# Autodesk Inventor assembly: Threaded Rod Actuator
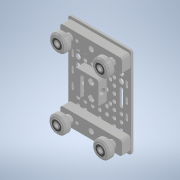
[picture p0: Inventor's stored thumbnail of the model, 180x180]
Saved by Autodesk Inventor 2020 (Build 240168000, 168)
## iProperties
Created: 2019-10-22
Part Number: Threaded Rod Actuator
Document SubType Name: Assembly
Designer: Johnson Ebenezer R
Author: Johnson Ebenezer R
## Documents named in this file (9)
- E:\My Tinkering Files\[2019-10-15][1330] Cam Controlled - PCB Paper's Fixture Hole - Punching Maching\Cam Controlled Paper Punching Machine (Prototype V2)\V-Slot Gantry Kit Universal (with gap for lead screw)\Gantry Kit (Vertical).iam
- E:\My Tinkering Files\[2019-10-15][1330] Cam Controlled - PCB Paper's Fixture Hole - Punching Maching\Cam Controlled Paper Punching Machine (Prototype V2)\V-Slot Gantry Kit Universal (with gap for lead screw)\V-Slot Gantry Plate 20-80mm.ipt
- E:\My Tinkering Files\[2019-10-15][1330] Cam Controlled - PCB Paper's Fixture Hole - Punching Maching\Cam Controlled Paper Punching Machine (Prototype V2)\V-Slot Gantry Kit Universal (with gap for lead screw)\8mm Acme Anti Backlash Nut Block.ipt
- E:\My Tinkering Files\[2019-10-15][1330] Cam Controlled - PCB Paper's Fixture Hole - Punching Maching\Cam Controlled Paper Punching Machine (Prototype V2)\V-Slot Gantry Kit Universal (with gap for lead screw)\Spacer Block.ipt
- E:\My Tinkering Files\[2019-10-15][1330] Cam Controlled - PCB Paper's Fixture Hole - Punching Maching\Cam Controlled Paper Punching Machine (Prototype V2)\V-Slot Gantry Kit Universal (with gap for lead screw)\Aluminum Spacer 6mm.ipt
- E:\My Tinkering Files\[2019-10-15][1330] Cam Controlled - PCB Paper's Fixture Hole - Punching Maching\Cam Controlled Paper Punching Machine (Prototype V2)\V-Slot Gantry Kit Universal (with gap for lead screw)\Eccentric Spacer 6mm.ipt
- E:\My Tinkering Files\[2019-10-15][1330] Cam Controlled - PCB Paper's Fixture Hole - Punching Maching\Cam Controlled Paper Punching Machine (Prototype V2)\V-Slot Gantry Kit Universal (with gap for lead screw)\Precision Shim 10 x 5 x 1.ipt
- E:\My Tinkering Files\[2019-10-15][1330] Cam Controlled - PCB Paper's Fixture Hole - Punching Maching\Cam Controlled Paper Punching Machine (Prototype V2)\V-Slot Gantry Kit Universal (with gap for lead screw)\Ball Bearing 5 x 16 x 5.ipt
- E:\My Tinkering Files\[2019-10-15][1330] Cam Controlled - PCB Paper's Fixture Hole - Punching Maching\Cam Controlled Paper Punching Machine (Prototype V2)\V-Slot Gantry Kit Universal (with gap for lead screw)\Xtreme Solid V Wheel.ipt
## Components (28 placed, 8 different names)
1. V-Slot Gantry Plate 20-80mm:1 — Mate:32, Mate:33, Mate:34, Mate:35, Flush:6, Mate:36, Mate:91, Mate:92, Mate:93
2. 8mm Acme Anti Backlash Nut Block:1 — Mate:91, Mate:92, Mate:93
3. Spacer Block:1 — Mate:32, Mate:33, Mate:34, Mate:37, Mate:38, Mate:39, Mate:40
4. Spacer Block:2 — Mate:35, Flush:6, Mate:36, Mate:51, Mate:52, Mate:53, Mate:54
5. Aluminum Spacer 6mm:1 — Mate:37, Mate:40, Mate:46, Mate:49
6. Aluminum Spacer 6mm:4 — Mate:38, Mate:39, Mate:45, Mate:50
7. Precision Shim 10 x 5 x 1:1 — Mate:46, Mate:49, Mate:58, Mate:66
8. Precision Shim 10 x 5 x 1:2 — Mate:45, Mate:50, Mate:57, Mate:65
9. Precision Shim 10 x 5 x 1:3 — Mate:67, Mate:72, Mate:75, Mate:79
10. Precision Shim 10 x 5 x 1:4 — Mate:68, Mate:71, Mate:76, Mate:80
11. Precision Shim 10 x 5 x 1:5 — Mate:55, Mate:62, Mate:64
12. Precision Shim 10 x 5 x 1:6 — Mate:56, Mate:60, Mate:61, Mate:63
13. Precision Shim 10 x 5 x 1:7 — Mate:69, Mate:74, Mate:77, Mate:82
14. Precision Shim 10 x 5 x 1:8 — Mate:70, Mate:73, Mate:78, Mate:81
15. Eccentric Spacer 6mm:1 — Mate:51, Mate:54, Mate:56, Mate:61
16. Eccentric Spacer 6mm:2 — Mate:52, Mate:53, Mate:55, Mate:59, Mate:62
17. Ball Bearing 5 x 16 x 5:1 — Mate:58, Mate:66, Mate:67, Mate:72, Mate:87
18. Ball Bearing 5 x 16 x 5:2 — Mate:75, Mate:79, Mate:83
19. Ball Bearing 5 x 16 x 5:3 — Mate:57, Mate:65, Mate:68, Mate:71, Mate:88
20. Ball Bearing 5 x 16 x 5:4 — Mate:76, Mate:80, Mate:84
21. Ball Bearing 5 x 16 x 5:5 — Mate:59, Mate:64, Mate:69, Mate:74, Mate:89
22. Ball Bearing 5 x 16 x 5:6 — Mate:77, Mate:82, Mate:85
23. Ball Bearing 5 x 16 x 5:7 — Mate:60, Mate:63, Mate:70, Mate:73, Mate:90
24. Ball Bearing 5 x 16 x 5:8 — Mate:78, Mate:81, Mate:86
25. Xtreme Solid V Wheel:1 — Mate:83, Mate:87
26. Xtreme Solid V Wheel:2 — Mate:84, Mate:88
27. Xtreme Solid V Wheel:3 — Mate:85, Mate:89
28. Xtreme Solid V Wheel:4 — Mate:86, Mate:90
## Relationships (57: Mate 56, Flush 1)
- Mate:32: V-Slot Gantry Plate 20-80mm:1 ↔ Spacer Block:1
- Mate:33: V-Slot Gantry Plate 20-80mm:1 ↔ Spacer Block:1
- Mate:34: V-Slot Gantry Plate 20-80mm:1 ↔ Spacer Block:1
- Mate:35: V-Slot Gantry Plate 20-80mm:1 ↔ Spacer Block:2
- Flush:6: V-Slot Gantry Plate 20-80mm:1 ↔ Spacer Block:2
- Mate:36: V-Slot Gantry Plate 20-80mm:1 ↔ Spacer Block:2
- Mate:37: Spacer Block:1 ↔ Aluminum Spacer 6mm:1
- Mate:38: Spacer Block:1 ↔ Aluminum Spacer 6mm:4
- Mate:39: Spacer Block:1 ↔ Aluminum Spacer 6mm:4
- Mate:40: Spacer Block:1 ↔ Aluminum Spacer 6mm:1
- Mate:45: Aluminum Spacer 6mm:4 ↔ Precision Shim 10 x 5 x 1:2
- Mate:46: Aluminum Spacer 6mm:1 ↔ Precision Shim 10 x 5 x 1:1
- Mate:49: Aluminum Spacer 6mm:1 ↔ Precision Shim 10 x 5 x 1:1
- Mate:50: Aluminum Spacer 6mm:4 ↔ Precision Shim 10 x 5 x 1:2
- Mate:51: Spacer Block:2 ↔ Eccentric Spacer 6mm:1
- Mate:52: Spacer Block:2 ↔ Eccentric Spacer 6mm:2
- Mate:53: Spacer Block:2 ↔ Eccentric Spacer 6mm:2
- Mate:54: Spacer Block:2 ↔ Eccentric Spacer 6mm:1
- Mate:55: Precision Shim 10 x 5 x 1:5 ↔ Eccentric Spacer 6mm:2
- Mate:56: Precision Shim 10 x 5 x 1:6 ↔ Eccentric Spacer 6mm:1
- Mate:57: Precision Shim 10 x 5 x 1:2 ↔ Ball Bearing 5 x 16 x 5:3
- Mate:58: Precision Shim 10 x 5 x 1:1 ↔ Ball Bearing 5 x 16 x 5:1
- Mate:59: Eccentric Spacer 6mm:2 ↔ Ball Bearing 5 x 16 x 5:5
- Mate:60: Precision Shim 10 x 5 x 1:6 ↔ Ball Bearing 5 x 16 x 5:7
- Mate:61: Precision Shim 10 x 5 x 1:6 ↔ Eccentric Spacer 6mm:1
- Mate:62: Precision Shim 10 x 5 x 1:5 ↔ Eccentric Spacer 6mm:2
- Mate:63: Precision Shim 10 x 5 x 1:6 ↔ Ball Bearing 5 x 16 x 5:7
- Mate:64: Precision Shim 10 x 5 x 1:5 ↔ Ball Bearing 5 x 16 x 5:5
- Mate:65: Precision Shim 10 x 5 x 1:2 ↔ Ball Bearing 5 x 16 x 5:3
- Mate:66: Precision Shim 10 x 5 x 1:1 ↔ Ball Bearing 5 x 16 x 5:1
- Mate:67: Precision Shim 10 x 5 x 1:3 ↔ Ball Bearing 5 x 16 x 5:1
- Mate:68: Precision Shim 10 x 5 x 1:4 ↔ Ball Bearing 5 x 16 x 5:3
- Mate:69: Precision Shim 10 x 5 x 1:7 ↔ Ball Bearing 5 x 16 x 5:5
- Mate:70: Precision Shim 10 x 5 x 1:8 ↔ Ball Bearing 5 x 16 x 5:7
- Mate:71: Precision Shim 10 x 5 x 1:4 ↔ Ball Bearing 5 x 16 x 5:3
- Mate:72: Precision Shim 10 x 5 x 1:3 ↔ Ball Bearing 5 x 16 x 5:1
- Mate:73: Precision Shim 10 x 5 x 1:8 ↔ Ball Bearing 5 x 16 x 5:7
- Mate:74: Precision Shim 10 x 5 x 1:7 ↔ Ball Bearing 5 x 16 x 5:5
- Mate:75: Precision Shim 10 x 5 x 1:3 ↔ Ball Bearing 5 x 16 x 5:2
- Mate:76: Precision Shim 10 x 5 x 1:4 ↔ Ball Bearing 5 x 16 x 5:4
- Mate:77: Precision Shim 10 x 5 x 1:7 ↔ Ball Bearing 5 x 16 x 5:6
- Mate:78: Precision Shim 10 x 5 x 1:8 ↔ Ball Bearing 5 x 16 x 5:8
- Mate:79: Precision Shim 10 x 5 x 1:3 ↔ Ball Bearing 5 x 16 x 5:2
- Mate:80: Precision Shim 10 x 5 x 1:4 ↔ Ball Bearing 5 x 16 x 5:4
- Mate:81: Precision Shim 10 x 5 x 1:8 ↔ Ball Bearing 5 x 16 x 5:8
- Mate:82: Precision Shim 10 x 5 x 1:7 ↔ Ball Bearing 5 x 16 x 5:6
- Mate:83: Ball Bearing 5 x 16 x 5:2 ↔ Xtreme Solid V Wheel:1
- Mate:84: Ball Bearing 5 x 16 x 5:4 ↔ Xtreme Solid V Wheel:2
- Mate:85: Ball Bearing 5 x 16 x 5:6 ↔ Xtreme Solid V Wheel:3
- Mate:86: Ball Bearing 5 x 16 x 5:8 ↔ Xtreme Solid V Wheel:4
- Mate:87: Ball Bearing 5 x 16 x 5:1 ↔ Xtreme Solid V Wheel:1
- Mate:88: Ball Bearing 5 x 16 x 5:3 ↔ Xtreme Solid V Wheel:2
- Mate:89: Ball Bearing 5 x 16 x 5:5 ↔ Xtreme Solid V Wheel:3
- Mate:90: Ball Bearing 5 x 16 x 5:7 ↔ Xtreme Solid V Wheel:4
- Mate:91: V-Slot Gantry Plate 20-80mm:1 ↔ 8mm Acme Anti Backlash Nut Block:1
- Mate:92: V-Slot Gantry Plate 20-80mm:1 ↔ 8mm Acme Anti Backlash Nut Block:1
- Mate:93: V-Slot Gantry Plate 20-80mm:1 ↔ 8mm Acme Anti Backlash Nut Block:1
